# Autodesk Inventor assembly: 01.02.03.00 - Braço esquerdo
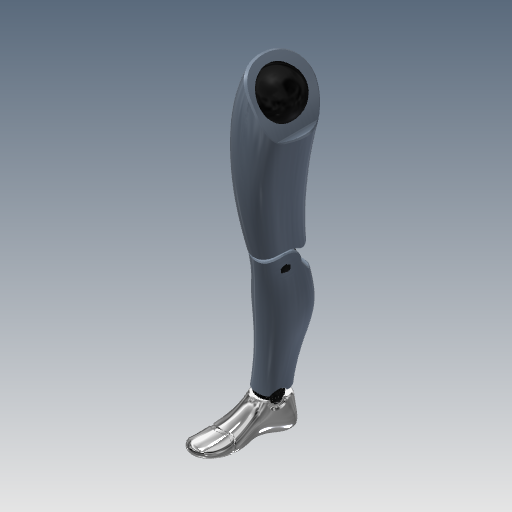
[picture p0: Inventor's stored thumbnail of the model, 512x512]
Saved by Autodesk Inventor 2018 (Build 220112000, 112)
## iProperties
Created: 2017-03-23
Part Number: 01.02.03.00 - Braço esquerdo
Document SubType Name: Assembly
Designer: Wesley Perez
Author: Wesley Perez
## Documents named in this file (4)
- C:\Users\Matt\robot\multibodySim\human\Corpo Humano - ADEBOTT Projetos\01.01.02.00 - Perna direita.iam
- C:\Users\Matt\robot\multibodySim\human\Corpo Humano - ADEBOTT Projetos\01.01.02.01 - Coxa direita.ipt
- C:\Users\Matt\robot\multibodySim\human\Corpo Humano - ADEBOTT Projetos\01.01.02.02 - Canela direita.ipt
- C:\Users\Matt\robot\multibodySim\human\Corpo Humano - ADEBOTT Projetos\01.01.02.03 - Pé direito.ipt
## Components (3 placed, 3 different names)
1. 01.01.02.01 - Coxa direita:1 — Alinhamento:1, Alinhamento:2, Alinhamento:3, Coincidência:1, Alinhamento:4
2. 01.01.02.02 - Canela direita:1 — Coincidência:1, Coincidência:2, Alinhamento:4, Alinhamento:5
3. 01.01.02.03 - Pé direito:1 — Coincidência:2, Alinhamento:5
## Relationships (7: Flush 5, Mate 2)
- Alinhamento:1 [Flush]: 01.01.02.01 - Coxa direita:1
- Alinhamento:2 [Flush]: 01.01.02.01 - Coxa direita:1
- Alinhamento:3 [Flush]: 01.01.02.01 - Coxa direita:1
- Coincidência:1 [Mate]: 01.01.02.01 - Coxa direita:1 ↔ 01.01.02.02 - Canela direita:1
- Coincidência:2 [Mate]: 01.01.02.02 - Canela direita:1 ↔ 01.01.02.03 - Pé direito:1
- Alinhamento:4 [Flush]: 01.01.02.01 - Coxa direita:1 ↔ 01.01.02.02 - Canela direita:1
- Alinhamento:5 [Flush]: 01.01.02.02 - Canela direita:1 ↔ 01.01.02.03 - Pé direito:1
